# Autodesk Inventor assembly: SampleHolder
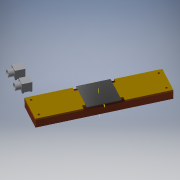
[picture p0: Inventor's stored thumbnail of the model, 180x180]
Saved by Autodesk Inventor 2017 SP1 (Build 210196100, 196)
## iProperties
Created: 2017-02-03
Part Number: SampleHolder
Document SubType Name: Assembly
Designer: Alex
Author: Alex
## Documents named in this file (5)
- C:\Users\Alex\Documents\git\CPWResonator\Inventor\SampleHolder.iam
- C:\Users\Alex\Documents\git\CPWResonator\Inventor\mount-base.ipt
- C:\Users\Alex\Documents\git\CPWResonator\Inventor\PCB-blank-20x20.ipt
- C:\Users\Alex\Documents\git\CPWResonator\Inventor\chip-blank-20x20.ipt
- C:\Users\Alex\Documents\git\CPWResonator\Inventor\Microwave Connector.ipt
## Components (5 placed, 4 different names)
1. mount-base:1 — Mate:1, Flush:1, Flush:2, Mate:4
2. PCB-blank-20x20:1 — Mate:1, Flush:1, Flush:2, Mate:2, Angle:1, Mate:4, Mate:5, Flush:3, Mate:6, Flush:4
3. chip-blank-20x20:1 — Mate:2, Mate:3, Angle:1
4. Microwave Connector:1 — Mate:5, Flush:3
5. Microwave Connector:2 — Mate:6, Flush:4
## Relationships (11: Mate 6, Flush 4, Angle 1)
- Mate:1: mount-base:1 ↔ PCB-blank-20x20:1
- Flush:1: mount-base:1 ↔ PCB-blank-20x20:1
- Flush:2: mount-base:1 ↔ PCB-blank-20x20:1
- Mate:2: PCB-blank-20x20:1 ↔ chip-blank-20x20:1
- Mate:3: chip-blank-20x20:1
- Angle:1 (0 deg): PCB-blank-20x20:1 ↔ chip-blank-20x20:1
- Mate:4: mount-base:1 ↔ PCB-blank-20x20:1
- Mate:5: PCB-blank-20x20:1 ↔ Microwave Connector:1
- Flush:3: PCB-blank-20x20:1 ↔ Microwave Connector:1
- Mate:6: PCB-blank-20x20:1 ↔ Microwave Connector:2
- Flush:4: PCB-blank-20x20:1 ↔ Microwave Connector:2
